# Autodesk Inventor assembly: outer
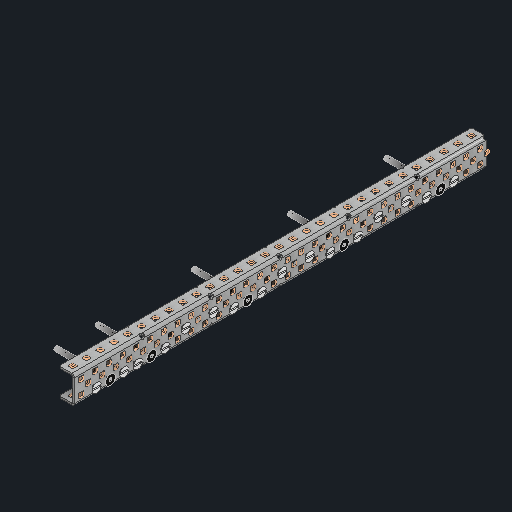
[picture p0: Inventor's stored thumbnail of the model, 512x512]
Saved by Autodesk Inventor 2025 (Build 290162000, 162)
## iProperties
Created: 2024-10-10
Part Number: outer
Document SubType Name: Assembly
Designer: Averey Ku
Author: Averey Ku
## Documents named in this file (4)
- D:\vex_robotics_high_stakes\hardware\cad\bots\high_stakes_v2\chassis_v2\drivebay\outer.iam
- D:\vex_robotics_high_stakes\hardware\cad\robpros_cad_lib\Structure\C Channel\Aluminum 1x2x1\Alu C 1x2x1x30.ipt
- D:\vex_robotics_high_stakes\hardware\cad\robpros_cad_lib\Quick Assemblies\bearing_flat_w_hardware.iam
- D:\vex_robotics_high_stakes\hardware\cad\robpros_cad_lib\Structure\Hardware\Screw Alloy Steel - Hex\ASScrew Hex Threaded 2.000.ipt
## Components (14 placed, 3 different names)
1. Alu C 1x2x1x30:1 — Insert:6, Mate:6, Insert:7, Mate:7, Insert:8, Insert:10, Insert:11, Mate:8
2. bearing_flat_w_hardware:8 [sub-assembly] — Insert:7, Mate:7
3. bearing_flat_w_hardware:9 [sub-assembly]
4. bearing_flat_w_hardware:10 [sub-assembly]
5. ASScrew Hex Threaded 2.000:5 — Insert:10
6. bearing_flat_w_hardware:7 [sub-assembly] — Insert:6, Mate:6
7. ASScrew Hex Threaded 2.000:10
8. bearing_flat_w_hardware:11 [sub-assembly]
9. ASScrew Hex Threaded 2.000:11
10. bearing_flat_w_hardware:12 [sub-assembly]
11. bearing_flat_w_hardware:13 [sub-assembly] — Insert:11, Mate:8
12. ASScrew Hex Threaded 2.000:1 — Insert:8
13. bearing_flat_w_hardware:14 [sub-assembly]
14. ASScrew Hex Threaded 2.000:12
## Component patterns: Motor Bearings (3 elements), Wheel Beariings (3 elements), (2 elements, first: bearing_flat_w_hardware:13 + ASScrew Hex Threaded 2.000:1)
## Relationships (8: Insert 5, Mate 3)
- Insert:6: Alu C 1x2x1x30:1 ↔ bearing_flat_w_hardware:7
- Mate:6: Alu C 1x2x1x30:1 ↔ bearing_flat_w_hardware:7
- Insert:7: Alu C 1x2x1x30:1 ↔ bearing_flat_w_hardware:8
- Mate:7: Alu C 1x2x1x30:1 ↔ bearing_flat_w_hardware:8
- Insert:8 (-1.5875 mm): Alu C 1x2x1x30:1 ↔ ASScrew Hex Threaded 2.000:1
- Insert:10 (-1.5875 mm): Alu C 1x2x1x30:1 ↔ ASScrew Hex Threaded 2.000:5
- Insert:11: Alu C 1x2x1x30:1 ↔ bearing_flat_w_hardware:13
- Mate:8: Alu C 1x2x1x30:1 ↔ bearing_flat_w_hardware:13
